# Autodesk Inventor assembly: Assembly
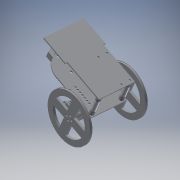
[picture p0: Inventor's stored thumbnail of the model, 180x180]
Saved by Autodesk Inventor 2016 (Build 200138000, 138)
## iProperties
Created: 2016-03-05
Part Number: Assembly
Document SubType Name: Assembly
Designer: mkepler
Author: mkepler
## Documents named in this file (6)
- C:\Users\mkepler\Google Drive\Michael Kepler\College\ECE\ECE 590\HW5\Physical Design\AUTOCAD part files\Assembly.iam
- C:\Users\mkepler\Google Drive\Michael Kepler\College\ECE\ECE 590\HW5\Physical Design\AUTOCAD part files\baseChassis322016.ipt
- C:\Users\mkepler\Google Drive\Michael Kepler\College\ECE\ECE 590\HW5\Physical Design\AUTOCAD part files\xl320Servo.ipt
- C:\Users\mkepler\Google Drive\Michael Kepler\College\ECE\ECE 590\HW5\Physical Design\AUTOCAD part files\wheel.ipt
- C:\Users\mkepler\Google Drive\Michael Kepler\College\ECE\ECE 590\HW5\Physical Design\AUTOCAD part files\peg.ipt
- C:\Users\mkepler\Google Drive\Michael Kepler\College\ECE\ECE 590\HW5\Physical Design\AUTOCAD part files\topChassis.ipt
## Components (9 placed, 5 different names)
1. baseChassis322016:1 — Insert:1, Insert:2, Insert:3, Insert:4, Insert:9, Insert:10, Insert:11
2. xl320Servo:1 — Insert:1, Insert:2, Insert:7, Insert:8
3. xl320Servo:2 — Insert:3, Insert:4, Insert:5, Insert:6
4. wheel:1 — Insert:5, Insert:6
5. wheel:2 — Insert:7, Insert:8
6. peg:1 — Insert:9, Mate:1
7. peg:2 — Insert:10
8. peg:3 — Insert:11, Insert:12
9. topChassis:1 — Insert:12, Mate:1
## Relationships (13: Insert 12, Mate 1)
- Insert:1: baseChassis322016:1 ↔ xl320Servo:1
- Insert:2: baseChassis322016:1 ↔ xl320Servo:1
- Insert:3: baseChassis322016:1 ↔ xl320Servo:2
- Insert:4: baseChassis322016:1 ↔ xl320Servo:2
- Insert:5: xl320Servo:2 ↔ wheel:1
- Insert:6: xl320Servo:2 ↔ wheel:1
- Insert:7: xl320Servo:1 ↔ wheel:2
- Insert:8: xl320Servo:1 ↔ wheel:2
- Insert:9: baseChassis322016:1 ↔ peg:1
- Insert:10: baseChassis322016:1 ↔ peg:2
- Insert:11: baseChassis322016:1 ↔ peg:3
- Insert:12: peg:3 ↔ topChassis:1
- Mate:1: peg:1 ↔ topChassis:1
